# Autodesk Inventor assembly: Camera_mount_v09
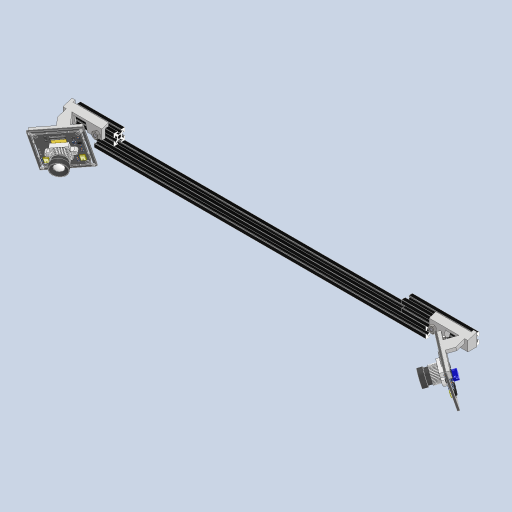
[picture p0: Inventor's stored thumbnail of the model, 512x512]
Saved by Autodesk Inventor 2024.4 (Build 284460000, 460)
## iProperties
Created: 2026-04-06
Part Number: Camera_mount_v09
Document SubType Name: Assembly
Designer: tooles01
Author: tooles01
## Documents named in this file (8)
- C:\Users\tooles01\NYU Langone Health Dropbox\Shannon Toole\Shannon_Dropbox\Mar lab\RFID\CAD\Camera_mount_angled\Camera_mount_v09.iam
- C:\Users\tooles01\NYU Langone Health Dropbox\Shannon Toole\Shannon_Dropbox\Mar lab\Inventor_Lib\100078 MB BE BL 300mm.ipt
- C:\Users\tooles01\Documents\Inventor\Content Center Files\R2024\en-US\AS 1112 (2)\AS 1112 - M2  Type 5.ipt
- C:\Users\tooles01\NYU Langone Health Dropbox\Shannon Toole\Shannon_Dropbox\Mar lab\RFID\CAD\Camera_mount_angled\mount_09.iam
- C:\Users\tooles01\NYU Langone Health Dropbox\Shannon Toole\Shannon_Dropbox\Mar lab\RFID\CAD\Camera_mount_angled\mount_09_mirror.iam
- C:\Users\tooles01\NYU Langone Health Dropbox\Shannon Toole\Shannon_Dropbox\Mar lab\Inventor_Lib\100078 MB BE BL 60mm.ipt
- C:\Users\tooles01\NYU Langone Health Dropbox\Shannon Toole\Shannon_Dropbox\Mar lab\Inventor_Lib\100078 MB BE BL 40mm.ipt
- C:\Users\tooles01\NYU Langone Health Dropbox\Shannon Toole\Shannon_Dropbox\Mar lab\RFID\CAD\lib\felt.ipt
## Components (7 placed, 7 different names)
1. felt:1 — long post flush to felt btm, long post to edge of felt, long post centered to felt
2. 100078 MB BE BL 300mm:1 — front post to large:end, front post to large:btm, front post to large:side, back post to large:end, back post to large:btm, back post to large:side, long post flush to felt btm, long post to edge of felt, long post centered to felt
3. 100078 MB BE BL 60mm:1 — front post to large:end, front post to large:btm, front post to large:side, angle piece to post top:1, angle piece flush to post:1, angle piece to post end:1
4. 100078 MB BE BL 40mm:1 — back post to large:end, back post to large:btm, back post to large:side, angle piece flush to post:2, angle piece to post end:2, angle piece to post top:2
5. mount_09:1 [sub-assembly] — camera nut to angle piece, angle piece flush to post:1, angle piece to post end:1, angle piece to post top:1
6. mount_09_mirror:1 [sub-assembly] — angle piece flush to post:2, angle piece to post end:2, angle piece to post top:2
7. AS 1112 (2) - Metric M2  Type 5:1 — camera nut to angle piece
## Relationships (16: Mate 10, Flush 5, Insert 1)
- camera nut to angle piece [Insert]: mount_09:1 ↔ AS 1112 (2) - Metric M2  Type 5:1
- angle piece flush to post:1 [Mate]: 100078 MB BE BL 60mm:1 ↔ mount_09:1
- angle piece to post end:1 [Mate]: 100078 MB BE BL 60mm:1 ↔ mount_09:1
- angle piece to post top:1 [Mate]: 100078 MB BE BL 60mm:1 ↔ mount_09:1
- angle piece flush to post:2 [Mate]: 100078 MB BE BL 40mm:1 ↔ mount_09_mirror:1
- angle piece to post end:2 [Mate]: 100078 MB BE BL 40mm:1 ↔ mount_09_mirror:1
- angle piece to post top:2 [Mate]: 100078 MB BE BL 40mm:1 ↔ mount_09_mirror:1
- front post to large:end [Flush] (-38 mm): 100078 MB BE BL 300mm:1 ↔ 100078 MB BE BL 60mm:1
- front post to large:btm [Mate]: 100078 MB BE BL 300mm:1 ↔ 100078 MB BE BL 60mm:1
- front post to large:side [Flush]: 100078 MB BE BL 300mm:1 ↔ 100078 MB BE BL 60mm:1
- back post to large:end [Flush] (-22 mm): 100078 MB BE BL 300mm:1 ↔ 100078 MB BE BL 40mm:1
- back post to large:btm [Mate]: 100078 MB BE BL 300mm:1 ↔ 100078 MB BE BL 40mm:1
- back post to large:side [Flush]: 100078 MB BE BL 300mm:1 ↔ 100078 MB BE BL 40mm:1
- long post flush to felt btm [Mate]: felt:1 ↔ 100078 MB BE BL 300mm:1
- long post to edge of felt [Flush] (90 mm): felt:1 ↔ 100078 MB BE BL 300mm:1
- long post centered to felt [Mate] (150 mm): felt:1 ↔ 100078 MB BE BL 300mm:1
